# Autodesk Inventor assembly: s-assy-unit-encoder
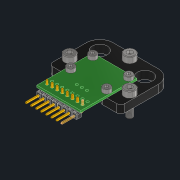
[picture p0: Inventor's stored thumbnail of the model, 180x180]
Saved by Autodesk Inventor 2022 (Build 260153000, 153)
## iProperties
Created: 2021-07-15
Part Number: s-assy-unit-encoder
Document SubType Name: Assembly
Designer: yuta0
Mass: 9.46827 g
Surface Area: 70.3785 cm^2
Volume: 5.20821 cm^3
Density: 1.81795 g/cm^3
Author: yuta0
## Documents named in this file (7)
- C:\Users\yuta0\Documents\GitHub\catchrobo_hardware\assy-robot\s-assy-unit-encoder.iam
- C:\Users\yuta0\Documents\GitHub\catchrobo_hardware\assy-robot\base29.ipt
- C:\Users\yuta0\Documents\GitHub\catchrobo_hardware\assy-robot\s-assy-AS5047P-TS_EK_AB.iam
- C:\Users\yuta0\Documents\GitHub\catchrobo_hardware\assy-robot\CB3-10.ipt
- C:\Users\yuta0\Documents\GitHub\catchrobo_hardware\assy-robot\CB2-4.ipt
- C:\Users\yuta0\Documents\GitHub\catchrobo_hardware\assy-robot\SB-203040.ipt
- C:\Users\yuta0\Documents\GitHub\catchrobo_hardware\assy-robot\Pin Header 1x8 TH Angle Pitch 2.54mm.ipt
## Components (14 placed, 6 different names)
1. unit-base5:1 — メイト:1, メイト:2, メイト:3, メイト:4, メイト:5, メイト:9, フラッシュ:1, メイト:12
2. s-assy-AS5047P-TS_EK_AB:1 [sub-assembly] — メイト:1, メイト:2, メイト:3, メイト:7, メイト:8, メイト:10, メイト:11, メイト:13, フラッシュ:3, メイト:14
3. Pin Header 1x8 TH Angle Pitch 2.54mm:1 — メイト:13, フラッシュ:3, メイト:14
4. CB3-10:1 — メイト:4, メイト:5
5. CB3-10:2
6. CB3-10:4
7. SB-203040:1 — メイト:9, フラッシュ:1, フラッシュ:2
8. CB2-4:2 — メイト:10, メイト:11
9. SB-203040:2 — メイト:12, フラッシュ:2
10. CB2-4:1 — メイト:7, メイト:8
11. SB-203040:3
12. CB2-4:3
13. SB-203040:4
14. CB2-4:4
## Component patterns: (4 elements, first: CB3-10:1), (2 elements, first: SB-203040:1 + CB2-4:2 + SB-203040:2 + CB2-4:1)
## Relationships (16: Mate 13, Flush 3)
- メイト:1 [Mate]: unit-base5:1 ↔ s-assy-AS5047P-TS_EK_AB:1
- メイト:2 [Mate]: unit-base5:1 ↔ s-assy-AS5047P-TS_EK_AB:1
- メイト:3 [Mate]: unit-base5:1 ↔ s-assy-AS5047P-TS_EK_AB:1
- メイト:4 [Mate]: unit-base5:1 ↔ CB3-10:1
- メイト:5 [Mate]: unit-base5:1 ↔ CB3-10:1
- メイト:7 [Mate]: s-assy-AS5047P-TS_EK_AB:1 ↔ CB2-4:1
- メイト:8 [Mate]: s-assy-AS5047P-TS_EK_AB:1 ↔ CB2-4:1
- メイト:9 [Mate]: unit-base5:1 ↔ SB-203040:1
- フラッシュ:1 [Flush]: unit-base5:1 ↔ SB-203040:1
- メイト:10 [Mate]: s-assy-AS5047P-TS_EK_AB:1 ↔ CB2-4:2
- メイト:11 [Mate]: s-assy-AS5047P-TS_EK_AB:1 ↔ CB2-4:2
- メイト:12 [Mate]: unit-base5:1 ↔ SB-203040:2
- フラッシュ:2 [Flush]: SB-203040:1 ↔ SB-203040:2
- メイト:13 [Mate]: s-assy-AS5047P-TS_EK_AB:1 ↔ Pin Header 1x8 TH Angle Pitch 2.54mm:1
- フラッシュ:3 [Flush] (0.85 mm): s-assy-AS5047P-TS_EK_AB:1 ↔ Pin Header 1x8 TH Angle Pitch 2.54mm:1
- メイト:14 [Mate] (-2.695 mm): s-assy-AS5047P-TS_EK_AB:1 ↔ Pin Header 1x8 TH Angle Pitch 2.54mm:1
